# Autodesk Inventor assembly: hodoscope
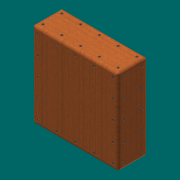
[picture p0: Inventor's stored thumbnail of the model, 180x180]
Saved by Autodesk Inventor 2016 SP1 (Build 200210100, 210)
## iProperties
Created: 2016-04-01
Part Number: hodoscope
Document SubType Name: Assembly
Designer: sawai
Author: sawai
## Documents named in this file (4)
- C:\Users\sawai\OneDrive\projects\modularHodoscope\hodoscope.iam
- C:\Users\sawai\OneDrive\projects\modularHodoscope\hodoscopeBare.iam
- C:\Users\sawai\OneDrive\projects\modularHodoscope\facing\frontBackFacing.iam
- C:\Users\sawai\OneDrive\projects\modularHodoscope\facing\sideFacing.iam
## Components (7 placed, 3 different names)
1. hodoscopeBare:1 [sub-assembly] — Mate:1, Mate:2, Flush:1, Flush:2, Flush:3, Flush:4, Mate:3, Flush:5, Mate:7, Mate:8, Flush:6, Mate:10
2. frontBackFacing:1 [sub-assembly] — Mate:2, Flush:1, Flush:2, Mate:4, Mate:6, Mate:12
3. frontBackFacing:2 [sub-assembly] — Mate:1, Flush:3, Flush:4, Mate:9
4. sideFacing:1 [sub-assembly] — Mate:3, Mate:4, Flush:5, Mate:5
5. sideFacing:2 [sub-assembly] — Mate:5, Mate:6, Mate:7, Mate:11
6. sideFacing:3 [sub-assembly] — Mate:8, Flush:6, Mate:9
7. sideFacing:4 [sub-assembly] — Mate:10, Mate:11, Mate:12
## Relationships (18: Mate 12, Flush 6)
- Mate:1: hodoscopeBare:1 ↔ frontBackFacing:2
- Mate:2: hodoscopeBare:1 ↔ frontBackFacing:1
- Flush:1: hodoscopeBare:1 ↔ frontBackFacing:1
- Flush:2: hodoscopeBare:1 ↔ frontBackFacing:1
- Flush:3: hodoscopeBare:1 ↔ frontBackFacing:2
- Flush:4: hodoscopeBare:1 ↔ frontBackFacing:2
- Mate:3: hodoscopeBare:1 ↔ sideFacing:1
- Mate:4: frontBackFacing:1 ↔ sideFacing:1
- Flush:5: hodoscopeBare:1 ↔ sideFacing:1
- Mate:5: sideFacing:1 ↔ sideFacing:2
- Mate:6: frontBackFacing:1 ↔ sideFacing:2
- Mate:7: hodoscopeBare:1 ↔ sideFacing:2
- Mate:8: hodoscopeBare:1 ↔ sideFacing:3
- Flush:6: hodoscopeBare:1 ↔ sideFacing:3
- Mate:9: frontBackFacing:2 ↔ sideFacing:3
- Mate:10: hodoscopeBare:1 ↔ sideFacing:4
- Mate:11: sideFacing:2 ↔ sideFacing:4
- Mate:12: frontBackFacing:1 ↔ sideFacing:4
